# Autodesk Inventor assembly: spool_stand
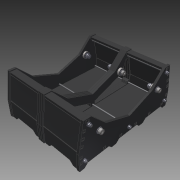
[picture p0: Inventor's stored thumbnail of the model, 180x180]
Saved by Autodesk Inventor 2014 (Build 180170000, 170)
## iProperties
Created: 2014-04-15
Part Number: spool_stand
Document SubType Name: Assembly
Designer: buben
Author: buben
## Documents named in this file (16)
- C:\Users\buben\Documents\GitHub\bspool\inventor_files\assemblies\spool_stand.iam
- C:\Users\buben\Documents\GitHub\bspool\inventor_files\parts\spool_stand_a.ipt
- C:\Users\buben\Documents\GitHub\bspool\inventor_files\parts\spool_stand_brace_bottom.ipt
- C:\Users\buben\Documents\GitHub\bspool\inventor_files\parts\spool_stand_brace_middle_a.ipt
- C:\Users\buben\Documents\GitHub\bspool\inventor_files\parts\spool_stand_brace_middle_b.ipt
- C:\Users\buben\Documents\GitHub\bspool\inventor_files\parts\spool_stand_brace_top.ipt
- C:\Users\buben\Documents\GitHub\bspool\inventor_files\parts\spool_stand_b.ipt
- C:\Users\buben\Documents\GitHub\bspool\inventor_files\3rd party components\bearing_608\Imported Components\608RS\608RS.ipt
- C:\Users\buben\Documents\GitHub\bspool\inventor_files\utils\washer_m5.ipt
- C:\Users\buben\Documents\Inventor\Content Center Files\R2014\en-US\ISO 7040\ISO 7040 - M5.ipt
- C:\Users\buben\Documents\GitHub\bspool\inventor_files\utils\threaded_rod_join.ipt
- C:\Users\buben\Documents\GitHub\bspool\inventor_files\utils\washer_m8.ipt
- C:\Users\buben\Documents\Inventor\Content Center Files\R2014\en-US\ISO 4762(2)\ISO 4762 - M8 x 25ISO.ipt
- C:\Users\buben\Documents\Inventor\Content Center Files\R2014\en-US\ISO 4762(2)\ISO 4762 - M8 x 45ISO.ipt
- C:\Users\buben\Documents\Inventor\Content Center Files\R2014\en-US\ISO 7040\ISO 7040 - M8.ipt
- C:\Users\buben\Documents\GitHub\bspool\inventor_files\parts\spool_stand_right.ipt
## Components (76 placed, 15 different names)
1. spool_stand_a:1 — Mate:1, Mate:2, Mate:3, Mate:4, Mate:5, Mate:6, Mate:8, Mate:11, Mate:12, Mate:13, Mate:14, Mate:15, Mate:16, Mate:17, Mate:18, Mate:19, Mate:20, Mate:21, Mate:22, Mate:23, Mate:24, Flush:1, Mate:56, Mate:57, Mate:58, Mate:69, Mate:70, Mate:83, Mate:84, Mate:85, Mate:86, Mate:87, Mate:88, Mate:89, Mate:90, Mate:91, Mate:92, Mate:108, Mate:134, Mate:135, Mate:136, Mate:137, Mate:154, Mate:155, Mate:156
2. spool_stand_brace_bottom:1 — Mate:4, Mate:5, Mate:6, Mate:31, Mate:32, Mate:33
3. spool_stand_brace_bottom:2 — Mate:40, Mate:41, Mate:42, Mate:55
4. spool_stand_brace_middle_a:1 — Mate:8, Mate:11, Mate:12
5. spool_stand_brace_middle_a:2 — Mate:46, Mate:47, Mate:48
6. spool_stand_brace_middle_a:4 — Mate:43, Mate:44, Mate:45
7. spool_stand_brace_middle_b:1 — Mate:13, Mate:14, Mate:15
8. spool_stand_brace_middle_b:2 — Mate:16, Mate:17, Mate:18
9. spool_stand_brace_middle_b:3 — Mate:49, Mate:50, Mate:51
10. spool_stand_brace_middle_b:4 — Mate:52, Mate:53, Mate:54
11. spool_stand_brace_top:1 — Mate:19, Mate:20, Mate:21
12. spool_stand_brace_top:2 — Mate:22, Mate:23, Mate:24
13. spool_stand_brace_top:3 — Mate:37, Mate:38, Mate:39
14. spool_stand_brace_top:4 — Mate:34, Mate:35, Mate:36
15. spool_stand_b:1 — Mate:25, Mate:26, Mate:27, Mate:31, Mate:32, Mate:33, Mate:63, Mate:64, Mate:65, Mate:66
16. spool_stand_b:2 — Mate:25, Mate:26, Mate:27, Mate:28, Mate:29, Mate:30
17. spool_stand_b:3 — Mate:28, Mate:29, Mate:30, Mate:34, Mate:35, Mate:36, Mate:37, Mate:38, Mate:39, Mate:40, Mate:41, Mate:42, Mate:43, Mate:44, Mate:45, Mate:46, Mate:47, Mate:48, Mate:49, Mate:50, Mate:51, Mate:52, Mate:53, Mate:54, Mate:59, Mate:60, Mate:67, Mate:68
18. spool_stand_right:1 — Mate:55, Flush:1, Mate:56, Mate:61, Mate:62, Mate:71, Mate:72, Mate:73, Mate:74, Mate:75, Mate:76, Mate:77, Mate:78, Mate:79, Mate:80, Mate:81, Mate:82, Mate:118, Mate:119, Mate:120, Mate:121
19. 608RS:1 — Mate:57, Mate:70, Mate:128, Mate:129
20. 608RS:2 — Mate:58, Mate:69, Mate:124, Mate:125
21. 608RS:3 — Mate:59, Mate:68, Mate:126, Mate:127
22. 608RS:4 — Mate:60, Mate:67, Mate:122, Mate:123
23. 608RS:5 — Mate:61, Mate:72, Mate:140, Mate:141
24. 608RS:6 — Mate:62, Mate:71, Mate:130, Mate:131
25. 608RS:7 — Mate:63, Mate:65, Mate:138, Mate:139
26. 608RS:8 — Mate:64, Mate:66, Mate:132, Mate:133
27. CSN 02 1702 B B 5,3:1 — Mate:75, Mate:76, Mate:111, Mate:112
28. CSN 02 1702 B B 5,3:2 — Mate:83, Mate:84, Mate:99, Mate:100
29. CSN 02 1702 B B 5,3:3 — Mate:73, Mate:74, Mate:109, Mate:110
30. CSN 02 1702 B B 5,3:4 — Mate:91, Mate:92, Mate:95, Mate:96
31. CSN 02 1702 B B 5,3:5 — Mate:85, Mate:86, Mate:97, Mate:98
32. CSN 02 1702 B B 5,3:6 — Mate:77, Mate:78, Mate:105, Mate:106
33. CSN 02 1702 B B 5,3:7 — Mate:79, Mate:80, Mate:101, Mate:102
34. CSN 02 1702 B B 5,3:8 — Mate:87, Mate:88, Mate:93, Mate:94
35. CSN 02 1702 B B 5,3:9 — Mate:81, Mate:82, Mate:103, Mate:104
36. CSN 02 1702 B B 5,3:10 — Mate:89, Mate:90, Mate:107
37. DIN EN ISO 7040 M5:1 — Mate:105, Mate:106
38. DIN EN ISO 7040 M5:2 — Mate:111, Mate:112
39. DIN EN ISO 7040 M5:3 — Mate:109, Mate:110
40. DIN EN ISO 7040 M5:4 — Mate:107, Mate:108, Mate:117, Flush:2
41. DIN EN ISO 7040 M5:5 — Mate:103, Mate:104
42. DIN EN ISO 7040 M5:6 — Mate:101, Mate:102
43. DIN EN ISO 7040 M5:7 — Mate:97, Mate:98, Mate:114, Flush:4
44. DIN EN ISO 7040 M5:8 — Mate:99, Mate:100, Mate:113, Flush:3
45. DIN EN ISO 7040 M5:9 — Mate:95, Mate:96, Mate:116, Flush:6
46. DIN EN ISO 7040 M5:10 — Mate:93, Mate:94, Mate:115, Flush:5
47. threaded_rod_join:1 — Mate:113, Flush:3
48. threaded_rod_join:2 — Mate:115, Flush:5
49. threaded_rod_join:3 — Mate:117, Flush:2
50. threaded_rod_join:4 — Mate:114, Flush:4
51. threaded_rod_join:5 — Mate:116, Flush:6
52. CSN 02 1702 B B 8,4:1 — Mate:126, Mate:127, Insert:6
53. CSN 02 1702 B B 8,4:4 — Mate:124, Mate:125, Mate:152
54. CSN 02 1702 B B 8,4:5 — Mate:122, Mate:123, Insert:5
55. CSN 02 1702 B B 8,4:6 — Mate:118, Mate:119, Insert:2
56. CSN 02 1702 B B 8,4:7 — Mate:120, Mate:121, Insert:1
57. CSN 02 1702 B B 8,4:8 — Mate:130, Mate:131, Mate:146
58. CSN 02 1702 B B 8,4:10 — Mate:138, Mate:139, Mate:142
59. CSN 02 1702 B B 8,4:11 — Mate:136, Mate:137, Insert:3
60. CSN 02 1702 B B 8,4:12 — Mate:132, Mate:133, Mate:148
61. CSN 02 1702 B B 8,4:13 — Mate:134, Mate:135, Insert:4
62. CSN 02 1702 B B 8,4:14 — Mate:128, Mate:129, Mate:150
63. CSN 02 1702 B B 8,4:15 — Mate:140, Mate:141, Mate:144
64. ISO 4762 M8 x 25:1 — Insert:4, Mate:153
65. ISO 4762 M8 x 25:2 — Insert:3, Mate:151
66. ISO 4762 M8 x 25:3 — Insert:2, Mate:147
67. ISO 4762 M8 x 25:4 — Insert:1, Mate:145
68. ISO 4762 M8 x 45:1 — Insert:6, Mate:149
69. ISO 4762 M8 x 45:2 — Insert:5, Mate:143
70. DIN EN ISO 7040 M8:1 — Mate:150, Mate:151
71. DIN EN ISO 7040 M8:2 — Mate:152, Mate:153
72. DIN EN ISO 7040 M8:3 — Mate:148, Mate:149
73. DIN EN ISO 7040 M8:4 — Mate:142, Mate:143
74. DIN EN ISO 7040 M8:5 — Mate:144, Mate:145
75. DIN EN ISO 7040 M8:6 — Mate:146, Mate:147
76. spool_stand_brace_middle_a:5 — Mate:154, Mate:155, Mate:156
## Relationships (165: Mate 153, Flush 6, Insert 6)
- Mate:1: spool_stand_a:1
- Mate:2: spool_stand_a:1
- Mate:3: spool_stand_a:1
- Mate:4: spool_stand_a:1 ↔ spool_stand_brace_bottom:1
- Mate:5: spool_stand_a:1 ↔ spool_stand_brace_bottom:1
- Mate:6: spool_stand_a:1 ↔ spool_stand_brace_bottom:1
- Mate:8: spool_stand_a:1 ↔ spool_stand_brace_middle_a:1
- Mate:11: spool_stand_a:1 ↔ spool_stand_brace_middle_a:1
- Mate:12: spool_stand_a:1 ↔ spool_stand_brace_middle_a:1
- Mate:13: spool_stand_a:1 ↔ spool_stand_brace_middle_b:1
- Mate:14: spool_stand_a:1 ↔ spool_stand_brace_middle_b:1
- Mate:15: spool_stand_a:1 ↔ spool_stand_brace_middle_b:1
- Mate:16: spool_stand_a:1 ↔ spool_stand_brace_middle_b:2
- Mate:17: spool_stand_a:1 ↔ spool_stand_brace_middle_b:2
- Mate:18: spool_stand_a:1 ↔ spool_stand_brace_middle_b:2
- Mate:19: spool_stand_a:1 ↔ spool_stand_brace_top:1
- Mate:20: spool_stand_a:1 ↔ spool_stand_brace_top:1
- Mate:21: spool_stand_a:1 ↔ spool_stand_brace_top:1
- Mate:22: spool_stand_a:1 ↔ spool_stand_brace_top:2
- Mate:23: spool_stand_a:1 ↔ spool_stand_brace_top:2
- Mate:24: spool_stand_a:1 ↔ spool_stand_brace_top:2
- Mate:25: spool_stand_b:1 ↔ spool_stand_b:2
- Mate:26: spool_stand_b:1 ↔ spool_stand_b:2
- Mate:27: spool_stand_b:1 ↔ spool_stand_b:2
- Mate:28: spool_stand_b:2 ↔ spool_stand_b:3
- Mate:29: spool_stand_b:2 ↔ spool_stand_b:3
- Mate:30: spool_stand_b:2 ↔ spool_stand_b:3
- Mate:31: spool_stand_brace_bottom:1 ↔ spool_stand_b:1
- Mate:32: spool_stand_brace_bottom:1 ↔ spool_stand_b:1
- Mate:33: spool_stand_brace_bottom:1 ↔ spool_stand_b:1
- Mate:34: spool_stand_brace_top:4 ↔ spool_stand_b:3
- Mate:35: spool_stand_brace_top:4 ↔ spool_stand_b:3
- Mate:36: spool_stand_brace_top:4 ↔ spool_stand_b:3
- Mate:37: spool_stand_brace_top:3 ↔ spool_stand_b:3
- Mate:38: spool_stand_brace_top:3 ↔ spool_stand_b:3
- Mate:39: spool_stand_brace_top:3 ↔ spool_stand_b:3
- Mate:40: spool_stand_brace_bottom:2 ↔ spool_stand_b:3
- Mate:41: spool_stand_brace_bottom:2 ↔ spool_stand_b:3
- Mate:42: spool_stand_brace_bottom:2 ↔ spool_stand_b:3
- Mate:43: spool_stand_brace_middle_a:4 ↔ spool_stand_b:3
- Mate:44: spool_stand_brace_middle_a:4 ↔ spool_stand_b:3
- Mate:45: spool_stand_brace_middle_a:4 ↔ spool_stand_b:3
- Mate:46: spool_stand_brace_middle_a:2 ↔ spool_stand_b:3
- Mate:47: spool_stand_brace_middle_a:2 ↔ spool_stand_b:3
- Mate:48: spool_stand_brace_middle_a:2 ↔ spool_stand_b:3
- Mate:49: spool_stand_brace_middle_b:3 ↔ spool_stand_b:3
- Mate:50: spool_stand_brace_middle_b:3 ↔ spool_stand_b:3
- Mate:51: spool_stand_brace_middle_b:3 ↔ spool_stand_b:3
- Mate:52: spool_stand_brace_middle_b:4 ↔ spool_stand_b:3
- Mate:53: spool_stand_brace_middle_b:4 ↔ spool_stand_b:3
- Mate:54: spool_stand_brace_middle_b:4 ↔ spool_stand_b:3
- Mate:55: spool_stand_brace_bottom:2 ↔ spool_stand_right:1
- Flush:1: spool_stand_a:1 ↔ spool_stand_right:1
- Mate:56: spool_stand_a:1 ↔ spool_stand_right:1
- Mate:57: spool_stand_a:1 ↔ 608RS:1
- Mate:58: spool_stand_a:1 ↔ 608RS:2
- Mate:59: spool_stand_b:3 ↔ 608RS:3
- Mate:60: spool_stand_b:3 ↔ 608RS:4
- Mate:61: spool_stand_right:1 ↔ 608RS:5
- Mate:62: spool_stand_right:1 ↔ 608RS:6
- Mate:63: spool_stand_b:1 ↔ 608RS:7
- Mate:64: spool_stand_b:1 ↔ 608RS:8
- Mate:65: spool_stand_b:1 ↔ 608RS:7
- Mate:66: spool_stand_b:1 ↔ 608RS:8
- Mate:67: spool_stand_b:3 ↔ 608RS:4
- Mate:68: spool_stand_b:3 ↔ 608RS:3
- Mate:69: spool_stand_a:1 ↔ 608RS:2
- Mate:70: spool_stand_a:1 ↔ 608RS:1
- Mate:71: spool_stand_right:1 ↔ 608RS:6
- Mate:72: spool_stand_right:1 ↔ 608RS:5
- Mate:73: spool_stand_right:1 ↔ CSN 02 1702 B B 5,3:3
- Mate:74: spool_stand_right:1 ↔ CSN 02 1702 B B 5,3:3
- Mate:75: spool_stand_right:1 ↔ CSN 02 1702 B B 5,3:1
- Mate:76: spool_stand_right:1 ↔ CSN 02 1702 B B 5,3:1
- Mate:77: spool_stand_right:1 ↔ CSN 02 1702 B B 5,3:6
- Mate:78: spool_stand_right:1 ↔ CSN 02 1702 B B 5,3:6
- Mate:79: spool_stand_right:1 ↔ CSN 02 1702 B B 5,3:7
- Mate:80: spool_stand_right:1 ↔ CSN 02 1702 B B 5,3:7
- Mate:81: spool_stand_right:1 ↔ CSN 02 1702 B B 5,3:9
- Mate:82: spool_stand_right:1 ↔ CSN 02 1702 B B 5,3:9
- Mate:83: spool_stand_a:1 ↔ CSN 02 1702 B B 5,3:2
- Mate:84: spool_stand_a:1 ↔ CSN 02 1702 B B 5,3:2
- Mate:85: spool_stand_a:1 ↔ CSN 02 1702 B B 5,3:5
- Mate:86: spool_stand_a:1 ↔ CSN 02 1702 B B 5,3:5
- Mate:87: spool_stand_a:1 ↔ CSN 02 1702 B B 5,3:8
- Mate:88: spool_stand_a:1 ↔ CSN 02 1702 B B 5,3:8
- Mate:89: spool_stand_a:1 ↔ CSN 02 1702 B B 5,3:10
- Mate:90: spool_stand_a:1 ↔ CSN 02 1702 B B 5,3:10
- Mate:91: spool_stand_a:1 ↔ CSN 02 1702 B B 5,3:4
- Mate:92: spool_stand_a:1 ↔ CSN 02 1702 B B 5,3:4
- Mate:93: CSN 02 1702 B B 5,3:8 ↔ DIN EN ISO 7040 M5:10
- Mate:94: CSN 02 1702 B B 5,3:8 ↔ DIN EN ISO 7040 M5:10
- Mate:95: CSN 02 1702 B B 5,3:4 ↔ DIN EN ISO 7040 M5:9
- Mate:96: CSN 02 1702 B B 5,3:4 ↔ DIN EN ISO 7040 M5:9
- Mate:97: CSN 02 1702 B B 5,3:5 ↔ DIN EN ISO 7040 M5:7
- Mate:98: CSN 02 1702 B B 5,3:5 ↔ DIN EN ISO 7040 M5:7
- Mate:99: CSN 02 1702 B B 5,3:2 ↔ DIN EN ISO 7040 M5:8
- Mate:100: CSN 02 1702 B B 5,3:2 ↔ DIN EN ISO 7040 M5:8
- Mate:101: CSN 02 1702 B B 5,3:7 ↔ DIN EN ISO 7040 M5:6
- Mate:102: CSN 02 1702 B B 5,3:7 ↔ DIN EN ISO 7040 M5:6
- Mate:103: CSN 02 1702 B B 5,3:9 ↔ DIN EN ISO 7040 M5:5
- Mate:104: CSN 02 1702 B B 5,3:9 ↔ DIN EN ISO 7040 M5:5
- Mate:105: CSN 02 1702 B B 5,3:6 ↔ DIN EN ISO 7040 M5:1
- Mate:106: CSN 02 1702 B B 5,3:6 ↔ DIN EN ISO 7040 M5:1
- Mate:107: CSN 02 1702 B B 5,3:10 ↔ DIN EN ISO 7040 M5:4
- Mate:108: spool_stand_a:1 ↔ DIN EN ISO 7040 M5:4
- Mate:109: CSN 02 1702 B B 5,3:3 ↔ DIN EN ISO 7040 M5:3
- Mate:110: CSN 02 1702 B B 5,3:3 ↔ DIN EN ISO 7040 M5:3
- Mate:111: CSN 02 1702 B B 5,3:1 ↔ DIN EN ISO 7040 M5:2
- Mate:112: CSN 02 1702 B B 5,3:1 ↔ DIN EN ISO 7040 M5:2
- Mate:113: DIN EN ISO 7040 M5:8 ↔ threaded_rod_join:1
- Mate:114: DIN EN ISO 7040 M5:7 ↔ threaded_rod_join:4
- Mate:115: DIN EN ISO 7040 M5:10 ↔ threaded_rod_join:2
- Mate:116: DIN EN ISO 7040 M5:9 ↔ threaded_rod_join:5
- Mate:117: DIN EN ISO 7040 M5:4 ↔ threaded_rod_join:3
- Flush:2 (-1 mm): DIN EN ISO 7040 M5:4 ↔ threaded_rod_join:3
- Flush:3 (-1 mm): DIN EN ISO 7040 M5:8 ↔ threaded_rod_join:1
- Flush:4 (-1 mm): DIN EN ISO 7040 M5:7 ↔ threaded_rod_join:4
- Flush:5 (-1 mm): DIN EN ISO 7040 M5:10 ↔ threaded_rod_join:2
- Flush:6 (-1 mm): DIN EN ISO 7040 M5:9 ↔ threaded_rod_join:5
- Mate:118: spool_stand_right:1 ↔ CSN 02 1702 B B 8,4:6
- Mate:119: spool_stand_right:1 ↔ CSN 02 1702 B B 8,4:6
- Mate:120: spool_stand_right:1 ↔ CSN 02 1702 B B 8,4:7
- Mate:121: spool_stand_right:1 ↔ CSN 02 1702 B B 8,4:7
- Mate:122: 608RS:4 ↔ CSN 02 1702 B B 8,4:5
- Mate:123: 608RS:4 ↔ CSN 02 1702 B B 8,4:5
- Mate:124: 608RS:2 ↔ CSN 02 1702 B B 8,4:4
- Mate:125: 608RS:2 ↔ CSN 02 1702 B B 8,4:4
- Mate:126: 608RS:3 ↔ CSN 02 1702 B B 8,4:1
- Mate:127: 608RS:3 ↔ CSN 02 1702 B B 8,4:1
- Mate:128: 608RS:1 ↔ CSN 02 1702 B B 8,4:14
- Mate:129: 608RS:1 ↔ CSN 02 1702 B B 8,4:14
- Mate:130: 608RS:6 ↔ CSN 02 1702 B B 8,4:8
- Mate:131: 608RS:6 ↔ CSN 02 1702 B B 8,4:8
- Mate:132: 608RS:8 ↔ CSN 02 1702 B B 8,4:12
- Mate:133: 608RS:8 ↔ CSN 02 1702 B B 8,4:12
- Mate:134: spool_stand_a:1 ↔ CSN 02 1702 B B 8,4:13
- Mate:135: spool_stand_a:1 ↔ CSN 02 1702 B B 8,4:13
- Mate:136: spool_stand_a:1 ↔ CSN 02 1702 B B 8,4:11
- Mate:137: spool_stand_a:1 ↔ CSN 02 1702 B B 8,4:11
- Mate:138: 608RS:7 ↔ CSN 02 1702 B B 8,4:10
- Mate:139: 608RS:7 ↔ CSN 02 1702 B B 8,4:10
- Mate:140: 608RS:5 ↔ CSN 02 1702 B B 8,4:15
- Mate:141: 608RS:5 ↔ CSN 02 1702 B B 8,4:15
- Insert:1: CSN 02 1702 B B 8,4:7 ↔ ISO 4762 M8 x 25:4
- Insert:2: CSN 02 1702 B B 8,4:6 ↔ ISO 4762 M8 x 25:3
- Insert:3: CSN 02 1702 B B 8,4:11 ↔ ISO 4762 M8 x 25:2
- Insert:4: CSN 02 1702 B B 8,4:13 ↔ ISO 4762 M8 x 25:1
- Insert:5: CSN 02 1702 B B 8,4:5 ↔ ISO 4762 M8 x 45:2
- Insert:6: CSN 02 1702 B B 8,4:1 ↔ ISO 4762 M8 x 45:1
- Mate:142: CSN 02 1702 B B 8,4:10 ↔ DIN EN ISO 7040 M8:4
- Mate:143: ISO 4762 M8 x 45:2 ↔ DIN EN ISO 7040 M8:4
- Mate:144: CSN 02 1702 B B 8,4:15 ↔ DIN EN ISO 7040 M8:5
- Mate:145: ISO 4762 M8 x 25:4 ↔ DIN EN ISO 7040 M8:5
- Mate:146: CSN 02 1702 B B 8,4:8 ↔ DIN EN ISO 7040 M8:6
- Mate:147: ISO 4762 M8 x 25:3 ↔ DIN EN ISO 7040 M8:6
- Mate:148: CSN 02 1702 B B 8,4:12 ↔ DIN EN ISO 7040 M8:3
- Mate:149: ISO 4762 M8 x 45:1 ↔ DIN EN ISO 7040 M8:3
- Mate:150: CSN 02 1702 B B 8,4:14 ↔ DIN EN ISO 7040 M8:1
- Mate:151: ISO 4762 M8 x 25:2 ↔ DIN EN ISO 7040 M8:1
- Mate:152: CSN 02 1702 B B 8,4:4 ↔ DIN EN ISO 7040 M8:2
- Mate:153: ISO 4762 M8 x 25:1 ↔ DIN EN ISO 7040 M8:2
- Mate:154: spool_stand_a:1 ↔ spool_stand_brace_middle_a:5
- Mate:155: spool_stand_a:1 ↔ spool_stand_brace_middle_a:5
- Mate:156: spool_stand_a:1 ↔ spool_stand_brace_middle_a:5
